# Autodesk Inventor assembly: Assemlby_OpenOxygen
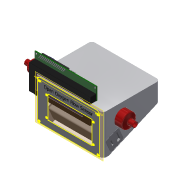
[picture p0: Inventor's stored thumbnail of the model, 180x180]
Saved by Autodesk Inventor 2019.4 (Build 234330000, 330)
## iProperties
Created: 2021-06-01
Part Number: Assemlby_OpenOxygen
Document SubType Name: Assembly
Designer: diederichbenedict
Author: diederichbenedict
## Documents named in this file (11)
- C:\Users\diederichbenedict\Dropbox\Dokumente\Promotion\PROJECTS\OXYGEN\INVENTOR\Assemlby_OpenOxygen.iam
- C:\Users\diederichbenedict\Dropbox\Dokumente\Promotion\PROJECTS\OXYGEN\INVENTOR\00_Sensirion_Flowsensor.ipt
- C:\Users\diederichbenedict\Dropbox\Dokumente\Promotion\PROJECTS\OXYGEN\INVENTOR\00_Arduino_LCD_I2Cstep.ipt
- C:\Users\diederichbenedict\Dropbox\Dokumente\Promotion\PROJECTS\OXYGEN\INVENTOR\00_ESP32.ipt
- C:\Users\diederichbenedict\Dropbox\Dokumente\Promotion\PROJECTS\OXYGEN\INVENTOR\00_Oxygen_Oxi.ipt
- C:\Users\diederichbenedict\Dropbox\Dokumente\Promotion\PROJECTS\OXYGEN\INVENTOR\00_LM286.ipt
- C:\Users\diederichbenedict\Dropbox\Dokumente\Promotion\PROJECTS\OXYGEN\INVENTOR\02_Connector_S.ipt
- C:\Users\diederichbenedict\Dropbox\Dokumente\Promotion\PROJECTS\OXYGEN\INVENTOR\03_OpenOxygen_Box.ipt
- C:\Users\diederichbenedict\Dropbox\Dokumente\Promotion\PROJECTS\OXYGEN\INVENTOR\00_Batterypack.ipt
- C:\Users\diederichbenedict\Dropbox\Dokumente\Promotion\PROJECTS\OXYGEN\INVENTOR\04_Adapterplate_Display.ipt
- C:\Users\diederichbenedict\Dropbox\Dokumente\Promotion\PROJECTS\OXYGEN\INVENTOR\02_Connector_T.ipt
## Components (10 placed, 10 different names)
1. 00_LM286:1
2. 00_Oxygen_Oxi:1
3. 03_OpenOxygen_Box:1 — Angle:4, Flush:7, Flush:8, Mate:1, Flush:9, Flush:10, Insert:1, Angle:5
4. 00_Batterypack:1 — Angle:4, Flush:7, Flush:8, Mate:1
5. 00_ESP32:1
6. 00_Arduino_LCD_I2Cstep:1
7. 04_Adapterplate_Display:1 — Flush:9, Flush:10
8. 00_Sensirion_Flowsensor:1 — Insert:1, Angle:5, Insert:2, Insert:3
9. 02_Connector_T:1 — Insert:3
10. 02_Connector_S:1 — Insert:2
## Relationships (10: Flush 4, Insert 3, Angle 2, Mate 1)
- Angle:4 (0 deg): 03_OpenOxygen_Box:1 ↔ 00_Batterypack:1
- Flush:7: 03_OpenOxygen_Box:1 ↔ 00_Batterypack:1
- Flush:8 (1 mm): 03_OpenOxygen_Box:1 ↔ 00_Batterypack:1
- Mate:1 (4 mm): 03_OpenOxygen_Box:1 ↔ 00_Batterypack:1
- Flush:9: 03_OpenOxygen_Box:1 ↔ 04_Adapterplate_Display:1
- Flush:10: 03_OpenOxygen_Box:1 ↔ 04_Adapterplate_Display:1
- Insert:1 (-4 mm): 03_OpenOxygen_Box:1 ↔ 00_Sensirion_Flowsensor:1
- Angle:5 (90 deg): 03_OpenOxygen_Box:1 ↔ 00_Sensirion_Flowsensor:1
- Insert:2 (-5 mm): 00_Sensirion_Flowsensor:1 ↔ 02_Connector_S:1
- Insert:3 (-5 mm): 00_Sensirion_Flowsensor:1 ↔ 02_Connector_T:1
